# Autodesk Inventor assembly: BottomPlate
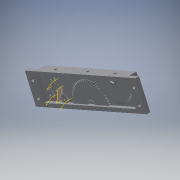
[picture p0: Inventor's stored thumbnail of the model, 180x180]
Saved by Autodesk Inventor 2016 (Build 200138000, 138)
## iProperties
Created: 2017-01-04
Part Number: BottomPlate
Document SubType Name: Assembly
Designer: james
Author: james
## Documents named in this file (5)
- C:\Users\james\Documents\Inventor\2017Ri3D\BottomPlate.iam
- C:\Users\james\Documents\Inventor\2017Ri3D\BottomWall.ipt
- C:\Users\james\Documents\Inventor\2017Ri3D\gear01.ipt
- C:\Users\james\Documents\Inventor\2017Ri3D\gear03.ipt
- C:\Users\james\Documents\Inventor\2017Ri3D\gear04.ipt
## Components (7 placed, 4 different names)
1. BottomWall:1 — Mate:1, Mate:2, Mate:3, Mate:4, Mate:5, Mate:6, Mate:7, Mate:8
2. gear01:1 — Mate:1, Mate:2
3. gear01:2 — Mate:3, Mate:4
4. gear03:1 — Mate:5
5. gear03:2 — Mate:7
6. gear03:3 — Mate:6
7. gear04:1 — Mate:8
## Relationships (8: Mate 8)
- Mate:1: BottomWall:1 ↔ gear01:1
- Mate:2: BottomWall:1 ↔ gear01:1
- Mate:3: BottomWall:1 ↔ gear01:2
- Mate:4: BottomWall:1 ↔ gear01:2
- Mate:5: BottomWall:1 ↔ gear03:1
- Mate:6: BottomWall:1 ↔ gear03:3
- Mate:7: BottomWall:1 ↔ gear03:2
- Mate:8: BottomWall:1 ↔ gear04:1
